# Autodesk Inventor assembly: moduleConnectorBracket
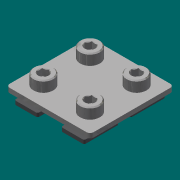
[picture p0: Inventor's stored thumbnail of the model, 180x180]
Saved by Autodesk Inventor 2016 SP1 (Build 200210100, 210)
## iProperties
Created: 2016-02-10
Part Number: moduleConnectorBracket
Document SubType Name: Assembly
Designer: Sawaiz
Author: Sawaiz
## Documents named in this file (4)
- C:\Users\sawaiz\oneDrive\projects\modularRichFrame\moduleConnectorBracket.iam
- C:\Users\sawaiz\OneDrive\projects\modularRICH\testMount\fingerHodoscope\SHPTSD5.ipt
- C:\Users\sawaiz\OneDrive\projects\modularRICH\testMount\hardware\m5TNut.ipt
- C:\Users\sawaiz\OneDrive\projects\modularRICH\testMount\hardware\m5x8.ipt
## Components (9 placed, 3 different names)
1. SHPTSD5:1 — Angle:1, Mate:10, Angle:5
2. m5x8:1
3. m5x8:2
4. m5x8:3
5. m5x8:4
6. m5TNut:1 — Flush:6, Angle:2
7. m5TNut:2 — Flush:4, Angle:1, Angle:2, Angle:3, Angle:5
8. m5TNut:3 — Flush:4, Flush:5, Angle:4
9. m5TNut:4 — Flush:5, Flush:6, Angle:3, Angle:4, Mate:10
## Relationships (21: Mate 10, Flush 6, Angle 5)
- [Mate]: SHPTSD5:1 ↔ m5x8:3
- [Mate]: SHPTSD5:1 ↔ m5x8:4
- [Mate]: SHPTSD5:1 ↔ m5x8:2
- [Mate]: SHPTSD5:1 ↔ m5x8:1
- [Flush]: m5x8:1 ↔ m5x8:4
- [Flush]: m5x8:3 ↔ m5x8:4
- [Flush]: m5x8:1 ↔ m5x8:2
- [Mate]: SHPTSD5:1 ↔ m5x8:3
- Flush:4: m5TNut:2 ↔ m5TNut:3
- Flush:5: m5TNut:3 ↔ m5TNut:4
- Flush:6: m5TNut:1 ↔ m5TNut:4
- Angle:1 (0 deg): SHPTSD5:1 ↔ m5TNut:2
- [Mate]: m5x8:3 ↔ m5TNut:2
- [Mate]: m5x8:2 ↔ m5TNut:4
- [Mate]: m5x8:1 ↔ m5TNut:3
- [Mate]: m5x8:4 ↔ m5TNut:1
- Angle:2 (0 deg): m5TNut:1 ↔ m5TNut:2
- Angle:3 (0 deg): m5TNut:2 ↔ m5TNut:4
- Angle:4 (0 deg): m5TNut:3 ↔ m5TNut:4
- Mate:10 (2 mm): SHPTSD5:1 ↔ m5TNut:4
- Angle:5 (0 deg): SHPTSD5:1 ↔ m5TNut:2
